# Autodesk Inventor assembly: assemblage
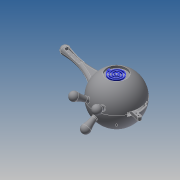
[picture p0: Inventor's stored thumbnail of the model, 180x180]
Saved by Autodesk Inventor 2017 (Build 210142000, 142)
## iProperties
Created: 2018-10-05
Part Number: assemblage
Document SubType Name: Assembly
Designer: Gilles Mottiez
Author: Gilles Mottiez
## Documents named in this file (15)
- C:\Users\Gilles Mottiez\Documents\HES\I5_6\PGA\inventor\assemblage.iam
- C:\Users\Gilles Mottiez\Documents\HES\I5_6\PGA\inventor\body_face.ipt
- C:\Users\Gilles Mottiez\Documents\HES\I5_6\PGA\inventor\body_dos.ipt
- C:\Users\Gilles Mottiez\Documents\HES\I5_6\PGA\inventor\pieds.ipt
- C:\Users\Gilles Mottiez\Documents\HES\I5_6\PGA\inventor\rpi3b.iam
- C:\Users\Gilles Mottiez\Documents\HES\I5_6\PGA\inventor\plateforme_rpi_servo.ipt
- C:\Users\Gilles Mottiez\Documents\HES\I5_6\PGA\inventor\MG90s_servo.ipt
- C:\Users\Gilles Mottiez\Documents\HES\I5_6\PGA\inventor\ressort.ipt
- C:\Users\Gilles Mottiez\Documents\HES\I5_6\PGA\inventor\palier_face.ipt
- palier_face.ipt
- C:\Users\Gilles Mottiez\Documents\HES\I5_6\PGA\inventor\arbre.ipt
- arbre.ipt
- C:\Users\Gilles Mottiez\Documents\HES\I5_6\PGA\inventor\bras_osc_dos.ipt
- bras_osc_dos.ipt
- C:\Users\Gilles Mottiez\Documents\HES\I5_6\PGA\inventor\bras_osc_front.ipt
## Components (13 placed, 10 different names)
1. body_face:1 — Logement:1, Logement:2, Logement:3, Logement:5, Placage:6, Placage:9, Logement:8, Affleurement:1
2. body_dos:1 — Logement:1, Logement:2, Logement:4
3. pieds:1 — Logement:3
4. pieds:2 — Logement:4
5. pieds:3 — Logement:5
6. rpi3b:1 [sub-assembly] — Logement:6, Logement:7
7. plateforme_rpi_servo:1 — Logement:6, Logement:7, Placage:3, Placage:4, Angle:1, Affleurement:1, Logement:10, Logement:11, Logement:12, Logement:13, Logement:14
8. MG90s_servo:1 — Placage:3, Placage:4, Angle:1
9. ressort:1 — Placage:6, Placage:9, Placage:10, Placage:11
10. palier_face:1 — Logement:8, Logement:9
11. arbre:1 — Logement:9, Placage:10, Placage:11, Logement:14
12. bras_osc_dos:1 — Logement:10, Logement:11
13. bras_osc_dos:2 — Logement:12, Logement:13
## Relationships (22: Insert 14, Mate 6, Angle 1, Flush 1)
- Logement:1 [Insert]: body_face:1 ↔ body_dos:1
- Logement:2 [Insert]: body_face:1 ↔ body_dos:1
- Logement:3 [Insert]: body_face:1 ↔ pieds:1
- Logement:4 [Insert]: body_dos:1 ↔ pieds:2
- Logement:5 [Insert]: body_face:1 ↔ pieds:3
- Logement:6 [Insert]: rpi3b:1 ↔ plateforme_rpi_servo:1
- Logement:7 [Insert]: rpi3b:1 ↔ plateforme_rpi_servo:1
- Placage:3 [Mate]: plateforme_rpi_servo:1 ↔ MG90s_servo:1
- Placage:4 [Mate]: plateforme_rpi_servo:1 ↔ MG90s_servo:1
- Angle:1 (180 deg): plateforme_rpi_servo:1 ↔ MG90s_servo:1
- Placage:6 [Mate]: body_face:1 ↔ ressort:1
- Placage:9 [Mate]: body_face:1 ↔ ressort:1
- Logement:8 [Insert]: body_face:1 ↔ palier_face:1
- Logement:9 [Insert]: palier_face:1 ↔ arbre:1
- Placage:10 [Mate]: ressort:1 ↔ arbre:1
- Affleurement:1 [Flush] (-5 mm): body_face:1 ↔ plateforme_rpi_servo:1
- Logement:10 [Insert]: plateforme_rpi_servo:1 ↔ bras_osc_dos:1
- Logement:11 [Insert]: plateforme_rpi_servo:1 ↔ bras_osc_dos:1
- Logement:12 [Insert]: plateforme_rpi_servo:1 ↔ bras_osc_dos:2
- Logement:13 [Insert]: plateforme_rpi_servo:1 ↔ bras_osc_dos:2
- Placage:11 [Mate]: ressort:1 ↔ arbre:1
- Logement:14 [Insert]: plateforme_rpi_servo:1 ↔ arbre:1
